# Autodesk Inventor assembly: ArmAssembly
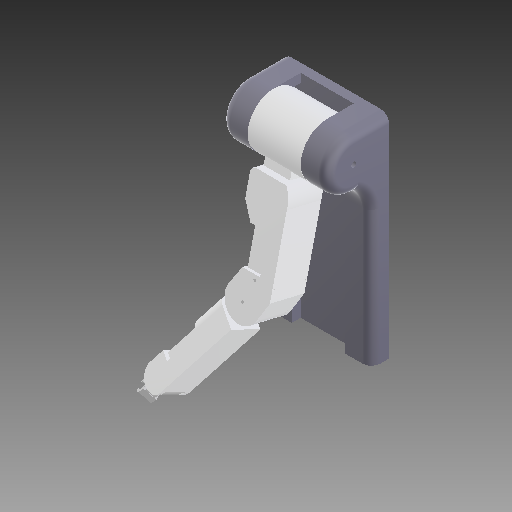
[picture p0: Inventor's stored thumbnail of the model, 512x512]
Saved by Autodesk Inventor 2017 SP1 (Build 210196100, 196)
## iProperties
Created: 2017-05-10
Part Number: ArmAssembly
Document SubType Name: Assembly
Designer: zallen
Author: zallen
## Documents named in this file (15)
- C:\Users\Zach\Documents\GitHub\cr-laundry-robot\src\Body\Arm Assembly\ArmAssembly.iam
- C:\Users\Zach\Documents\GitHub\cr-laundry-robot\src\Body\Arm Assembly\Part1.ipt
- C:\Users\Zach\Documents\GitHub\cr-laundry-robot\src\Body\Arm Assembly\Part2.ipt
- C:\Users\Zach\Documents\GitHub\cr-laundry-robot\src\Body\Arm Assembly\Part3.ipt
- C:\Users\Zach\Documents\GitHub\cr-laundry-robot\src\Body\Arm Assembly\Part4.ipt
- C:\Users\Zach\Documents\GitHub\cr-laundry-robot\src\Body\Arm Assembly\Part5.ipt
- C:\Users\Zach\Documents\GitHub\cr-laundry-robot\src\Body\Arm Assembly\Part6.ipt
- C:\Users\Zach\Documents\GitHub\cr-laundry-robot\src\Body\Arm Assembly\Part7.ipt
- C:\Users\Zach\Documents\GitHub\cr-laundry-robot\src\Body\Arm Assembly\Part8.ipt
- C:\Users\Zach\Documents\GitHub\cr-laundry-robot\lib\Stepper Motor\Двигатель.ipt
- C:\Users\Zach\Documents\GitHub\cr-laundry-robot\src\Body\Arm Assembly\ArmAssembly\Design Accelerator\Spur Gears2.iam
- C:\Users\Zach\Documents\GitHub\cr-laundry-robot\src\Body\Arm Assembly\ArmAssembly\Design Accelerator\Spur Gears3.iam
- C:\Users\Zach\Documents\GitHub\cr-laundry-robot\src\Body\Arm Assembly\Part10.ipt
- C:\Users\Zach\Documents\GitHub\cr-laundry-robot\src\Body\Arm Assembly\Part11.ipt
- C:\Users\Zach\Documents\GitHub\cr-laundry-robot\src\Body\Arm Assembly\Part12.ipt
## Components (18 placed, 13 different names)
1. Part1:1 — Mate:1, Mate:29, Mate:30, Mate:31, Mate:32, Mate:33, Rotational:12
2. Part2:1 — Mate:1, Rotational:12, Mate:34, Mate:35, Mate:36, Mate:37, Mate:38, Rotational:13
3. Part3:1 — Mate:38, Rotational:13, Mate:39, Rotational:16, Mate:41, Mate:42, Mate:43, Mate:47, Mate:49, Mate:51, Mate:52, Mate:55, Mate:56, Mate:57, Mate:58, Mate:59, Mate:60, Mate:61, Mate:62
4. Part4:1 — Mate:39, Mate:40, Rotational:15, Rotational:16
5. Part5:1 — Mate:8, Rotational:8, Mate:40, Rotational:15
6. Part6:1 — Mate:8, Mate:9, Rotational:8, Rotational:9
7. Part7:1 — Mate:9, Rotational:9, Mate:10, Rotational:10, Mate:11, Rotational:11
8. Part8:1 — Mate:10, Rotational:10
9. Part8:2 — Mate:11, Rotational:11
10. Двигатель:2 — Mate:29, Mate:30, Mate:31, Mate:32, Mate:33
11. Двигатель:3 — Mate:34, Mate:35, Mate:36, Mate:37
12. Двигатель:4 — Mate:41, Mate:42, Mate:43, Mate:46
13. Spur Gears:1 [sub-assembly] — Mate:46, Mate:47
14. Spur Gears:2 [sub-assembly] — Mate:49
15. Part10:1 — Mate:51, Mate:54
16. Part11:1 — Mate:52, Mate:54, Mate:55, Mate:56
17. Part11:2 — Mate:57, Mate:58, Mate:59
18. Part12:1 — Mate:60, Mate:61, Mate:62
## Relationships (42: Mate 34, RevoluteJoint 8)
- Mate:1: Part1:1 ↔ Part2:1
- Mate:8: Part5:1 ↔ Part6:1
- Mate:9: Part6:1 ↔ Part7:1
- Rotational:8 [RevoluteJoint]: Part5:1 ↔ Part6:1
- Rotational:9 [RevoluteJoint]: Part6:1 ↔ Part7:1
- Mate:10: Part7:1 ↔ Part8:1
- Rotational:10 [RevoluteJoint]: Part7:1 ↔ Part8:1
- Mate:11: Part7:1 ↔ Part8:2
- Rotational:11 [RevoluteJoint]: Part7:1 ↔ Part8:2
- Mate:29: Part1:1 ↔ Двигатель:2
- Mate:30: Part1:1 ↔ Двигатель:2
- Mate:31: Part1:1 ↔ Двигатель:2
- Mate:32: Part1:1 ↔ Двигатель:2
- Mate:33: Part1:1 ↔ Двигатель:2
- Rotational:12 [RevoluteJoint]: Part1:1 ↔ Part2:1
- Mate:34: Part2:1 ↔ Двигатель:3
- Mate:35: Part2:1 ↔ Двигатель:3
- Mate:36: Part2:1 ↔ Двигатель:3
- Mate:37: Part2:1 ↔ Двигатель:3
- Mate:38: Part2:1 ↔ Part3:1
- Rotational:13 [RevoluteJoint]: Part2:1 ↔ Part3:1
- Mate:39: Part3:1 ↔ Part4:1
- Mate:40: Part4:1 ↔ Part5:1
- Rotational:15 [RevoluteJoint]: Part4:1 ↔ Part5:1
- Rotational:16 [RevoluteJoint]: Part3:1 ↔ Part4:1
- Mate:41: Part3:1 ↔ Двигатель:4
- Mate:42: Part3:1 ↔ Двигатель:4
- Mate:43: Part3:1 ↔ Двигатель:4
- Mate:46: Двигатель:4 ↔ Spur Gears:1
- Mate:47: Part3:1 ↔ Spur Gears:1
- Mate:49: Part3:1 ↔ Spur Gears:2
- Mate:51: Part3:1 ↔ Part10:1
- Mate:52: Part3:1 ↔ Part11:1
- Mate:54: Part10:1 ↔ Part11:1
- Mate:55: Part3:1 ↔ Part11:1
- Mate:56: Part3:1 ↔ Part11:1
- Mate:57: Part3:1 ↔ Part11:2
- Mate:58: Part3:1 ↔ Part11:2
- Mate:59: Part3:1 ↔ Part11:2
- Mate:60: Part3:1 ↔ Part12:1
- Mate:61: Part3:1 ↔ Part12:1
- Mate:62: Part3:1 ↔ Part12:1
